# Autodesk Inventor assembly: Structure
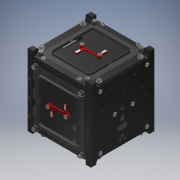
[picture p0: Inventor's stored thumbnail of the model, 180x180]
Saved by Autodesk Inventor 2018 (Build 220112000, 112)
## iProperties
Created: 2019-03-30
Part Number: Structure
Document SubType Name: Assembly
Designer: Bradley
Author: Bradley
## Documents named in this file (17)
- C:\Users\Bradley\Documents\GitHub\CougSat1-Hardware\CougSat1-Structure\CADModel\Imported\Structure.iam
- C:\Users\Bradley\Documents\GitHub\CougSat1-Hardware\CougSat1-Structure\CADModel\Imported\Structure_+X.ipt
- C:\Users\Bradley\Documents\GitHub\CougSat1-Hardware\CougSat1-Structure\CADModel\Imported\Structure_-X.ipt
- C:\Users\Bradley\Documents\GitHub\CougSat1-Hardware\CougSat1-Structure\CADModel\Imported\Structure_+Z.ipt
- C:\Users\Bradley\Documents\GitHub\CougSat1-Hardware\CougSat1-Structure\CADModel\Imported\Structure_Y.ipt
- C:\Users\Bradley\Documents\GitHub\CougSat1-Hardware\CougSat1-Structure\CADModel\Imported\Structure_-Z.ipt
- C:\Users\Bradley\Documents\GitHub\CougSat1-Hardware\CougSat1-Structure\CADModel\Imported\Structure_SolarPanelHeatsink.ipt
- C:\Users\Bradley\Documents\GitHub\CougSat1-Hardware\CougSat1-Structure\CADModel\Imported\Structure_MagnetorquerForm.ipt
- C:\Users\Bradley\Documents\GitHub\Resources\SupplierDocuments\48 - Hardware\48-0361\48-0361.ipt
- C:\Users\Bradley\Documents\GitHub\Resources\SupplierDocuments\48 - Hardware\48-0340\48-0340.ipt
- C:\Users\Bradley\Documents\GitHub\Resources\SupplierDocuments\48 - Hardware\48-0350\48-0350.ipt
- C:\Users\Bradley\Documents\GitHub\Resources\SupplierDocuments\48 - Hardware\48-0300\48-0300.ipt
- C:\Users\Bradley\Documents\GitHub\Resources\SupplierDocuments\48 - Hardware\48-0001\48-0001.ipt
- C:\Users\Bradley\Documents\GitHub\Resources\SupplierDocuments\48 - Hardware\48-0381\48-0381.ipt
- C:\Users\Bradley\Documents\GitHub\Resources\SupplierDocuments\48 - Hardware\48-0362\48-0362.ipt
- C:\Users\Bradley\Documents\GitHub\Resources\SupplierDocuments\48 - Hardware\48-03A1\48-03A1.ipt
- C:\Users\Bradley\Documents\GitHub\Resources\SupplierDocuments\49 - Electromechanical\49-0006\49-0006.ipt
## Components (81 placed, 16 different names)
1. 49-0006:3 — Mate:6, Flush:1, Flush:2
2. 49-0006:2 — Mate:4, Flush:3
3. 49-0006:1 — Mate:5, Flush:2, Flush:3
4. 48-0001:1 — Insert:27
5. 48-0001:2 — Insert:28
6. 48-0300:1 — Insert:29, Insert:30
7. 48-0300:10 — Insert:42
8. 48-0300:11 — Insert:38
9. 48-0300:12 — Insert:54
10. 48-0300:2 — Insert:53
11. 48-0300:3 — Insert:51
12. 48-0300:4 — Insert:52
13. 48-0300:5 — Insert:83, Insert:87
14. 48-0300:6 — Insert:84, Insert:88
15. 48-0300:7 — Insert:85, Insert:90
16. 48-0300:8 — Insert:86, Insert:89
17. 48-0300:9 — Insert:41
18. 48-0340:1 — Insert:77
19. 48-0340:10 — Insert:90
20. 48-0340:2 — Insert:89
21. 48-0340:3 — Insert:78
22. 48-0340:4 — Insert:79
23. 48-0340:5 — Insert:80
24. 48-0340:6 — Insert:81
25. 48-0340:7 — Insert:82
26. 48-0340:8 — Insert:87
27. 48-0340:9 — Insert:88
28. 48-0350:1 — Insert:43
29. 48-0350:2 — Insert:44
30. 48-0350:3 — Insert:45
31. 48-0350:4 — Insert:46
32. 48-0350:5 — Insert:58
33. 48-0350:6 — Insert:57
34. 48-0350:7 — Insert:55
35. 48-0350:8 — Insert:56
36. 48-0362:1 — Insert:91
37. 48-0362:2 — Insert:92
38. 48-0362:3 — Insert:94
39. 48-0362:4 — Insert:93
40. 48-0361:1 — Insert:29
41. 48-0361:2
42. 48-0361:3
43. 48-0361:4
44. 48-0361:5
45. 48-0361:6
46. 48-0361:7
47. 48-0361:8
48. 48-0381:1 — Insert:59
49. 48-0381:18 — Insert:75
50. 48-0381:2 — Insert:60
51. 48-0381:3 — Insert:63
52. 48-0381:4 — Insert:64
53. 48-0381:5 — Insert:61
54. 48-0381:6 — Insert:62
55. 48-0381:7 — Insert:65
56. 48-0381:8 — Insert:66
57. 48-0381:9 — Insert:67
58. 48-0381:10 — Insert:68
59. 48-0381:11 — Insert:69
60. 48-0381:12 — Insert:70
61. 48-0381:13 — Insert:71
62. 48-0381:14 — Insert:72
63. 48-0381:15 — Insert:74
64. 48-0381:16 — Insert:73
65. 48-0381:17 — Insert:76
66. 48-03A1:1 — Insert:95
67. 48-03A1:2 — Insert:96
68. Structure_+X:1 — Mate:1, Mate:2, Insert:1, Insert:2, Mate:3, Insert:9, Insert:10, Insert:27, Insert:77, Insert:78, Insert:79, Insert:80, Insert:81, Insert:82
69. Structure_+Z:1 — Insert:1, Insert:2, Insert:3, Insert:4, Insert:5, Insert:6, Insert:7, Insert:8, Insert:13, Insert:14, Insert:23, Insert:24, Insert:30, Insert:38, Insert:41, Insert:42, Insert:43, Insert:44, Insert:45, Insert:46
70. Structure_-X:1 — Insert:7, Insert:8, Insert:17, Insert:18, Insert:21, Insert:22, Insert:28, Mate:4, Mate:5, Mate:6, Flush:1
71. Structure_-Z:1 — Insert:9, Insert:10, Insert:51, Insert:52, Insert:53, Insert:54, Insert:55, Insert:56, Insert:57, Insert:58, Insert:83, Insert:84, Insert:85, Insert:86
72. Structure_MagnetorquerForm:1 — Insert:19, Insert:20, Insert:59, Insert:60, Insert:63, Insert:64
73. Structure_MagnetorquerForm:2 — Insert:21, Insert:22, Insert:91, Insert:92, Insert:93, Insert:94
74. Structure_MagnetorquerForm:3 — Insert:23, Insert:24, Insert:71, Insert:72, Insert:75, Insert:76
75. Structure_MagnetorquerForm:4 — Insert:25, Insert:26, Insert:65, Insert:66, Insert:69, Insert:70
76. Structure_SolarPanelHeatsink:1 — Insert:13, Insert:14, Insert:73, Insert:74
77. Structure_SolarPanelHeatsink:2 — Insert:11, Insert:12, Insert:61, Insert:62
78. Structure_SolarPanelHeatsink:3 — Insert:17, Insert:18, Insert:95, Insert:96
79. Structure_SolarPanelHeatsink:4 — Insert:15, Insert:16, Insert:67, Insert:68
80. Structure_Y:1 — Insert:3, Insert:4, Insert:11, Insert:12, Insert:19, Insert:20
81. Structure_Y:2 — Insert:5, Insert:6, Insert:15, Insert:16, Insert:25, Insert:26
## Relationships (99: Insert 90, Mate 6, Flush 3)
- Mate:1 (50 mm): Structure_+X:1
- Mate:2 (-49 mm): Structure_+X:1
- Insert:1: Structure_+X:1 ↔ Structure_+Z:1
- Insert:2: Structure_+X:1 ↔ Structure_+Z:1
- Insert:3: Structure_+Z:1 ↔ Structure_Y:1
- Insert:4: Structure_+Z:1 ↔ Structure_Y:1
- Insert:5: Structure_+Z:1 ↔ Structure_Y:2
- Insert:6: Structure_+Z:1 ↔ Structure_Y:2
- Insert:7: Structure_+Z:1 ↔ Structure_-X:1
- Insert:8: Structure_+Z:1 ↔ Structure_-X:1
- Mate:3 (50 mm): Structure_+X:1
- Insert:9: Structure_+X:1 ↔ Structure_-Z:1
- Insert:10: Structure_+X:1 ↔ Structure_-Z:1
- Insert:11: Structure_SolarPanelHeatsink:2 ↔ Structure_Y:1
- Insert:12: Structure_SolarPanelHeatsink:2 ↔ Structure_Y:1
- Insert:13: Structure_+Z:1 ↔ Structure_SolarPanelHeatsink:1
- Insert:14: Structure_+Z:1 ↔ Structure_SolarPanelHeatsink:1
- Insert:15: Structure_SolarPanelHeatsink:4 ↔ Structure_Y:2
- Insert:16: Structure_SolarPanelHeatsink:4 ↔ Structure_Y:2
- Insert:17: Structure_-X:1 ↔ Structure_SolarPanelHeatsink:3
- Insert:18: Structure_-X:1 ↔ Structure_SolarPanelHeatsink:3
- Insert:19: Structure_MagnetorquerForm:1 ↔ Structure_Y:1
- Insert:20: Structure_MagnetorquerForm:1 ↔ Structure_Y:1
- Insert:21: Structure_-X:1 ↔ Structure_MagnetorquerForm:2
- Insert:22: Structure_-X:1 ↔ Structure_MagnetorquerForm:2
- Insert:23: Structure_+Z:1 ↔ Structure_MagnetorquerForm:3
- Insert:24: Structure_+Z:1 ↔ Structure_MagnetorquerForm:3
- Insert:25: Structure_MagnetorquerForm:4 ↔ Structure_Y:2
- Insert:26: Structure_MagnetorquerForm:4 ↔ Structure_Y:2
- Insert:27: 48-0001:1 ↔ Structure_+X:1
- Insert:28: 48-0001:2 ↔ Structure_-X:1
- Insert:29: 48-0300:1 ↔ 48-0361:1
- Insert:30: 48-0300:1 ↔ Structure_+Z:1
- [Insert]: 48-0300:9 ↔ 48-0361:5
- [Insert]: 48-0300:10 ↔ 48-0361:6
- [Insert]: 48-0300:11 ↔ 48-0361:7
- Insert:38: 48-0300:11 ↔ Structure_+Z:1
- Insert:41: 48-0300:9 ↔ Structure_+Z:1
- Insert:42: 48-0300:10 ↔ Structure_+Z:1
- Insert:43: 48-0350:1 ↔ Structure_+Z:1
- Insert:44: 48-0350:2 ↔ Structure_+Z:1
- Insert:45: 48-0350:3 ↔ Structure_+Z:1
- Insert:46: 48-0350:4 ↔ Structure_+Z:1
- [Insert]: 48-0300:12 ↔ 48-0361:8
- [Insert]: 48-0300:2 ↔ 48-0361:2
- [Insert]: 48-0300:3 ↔ 48-0361:3
- [Insert]: 48-0300:4 ↔ 48-0361:4
- Insert:51: 48-0300:3 ↔ Structure_-Z:1
- Insert:52: 48-0300:4 ↔ Structure_-Z:1
- Insert:53: 48-0300:2 ↔ Structure_-Z:1
- Insert:54: 48-0300:12 ↔ Structure_-Z:1
- Insert:55: 48-0350:7 ↔ Structure_-Z:1
- Insert:56: 48-0350:8 ↔ Structure_-Z:1
- Insert:57: 48-0350:6 ↔ Structure_-Z:1
- Insert:58: 48-0350:5 ↔ Structure_-Z:1
- Insert:59 (1 mm): 48-0381:1 ↔ Structure_MagnetorquerForm:1
- Insert:60 (1 mm): 48-0381:2 ↔ Structure_MagnetorquerForm:1
- Insert:61 (1 mm): 48-0381:5 ↔ Structure_SolarPanelHeatsink:2
- Insert:62 (1 mm): 48-0381:6 ↔ Structure_SolarPanelHeatsink:2
- Insert:63 (1 mm): 48-0381:3 ↔ Structure_MagnetorquerForm:1
- Insert:64 (1 mm): 48-0381:4 ↔ Structure_MagnetorquerForm:1
- Insert:65 (1 mm): 48-0381:7 ↔ Structure_MagnetorquerForm:4
- Insert:66 (1 mm): 48-0381:8 ↔ Structure_MagnetorquerForm:4
- Insert:67 (1 mm): 48-0381:9 ↔ Structure_SolarPanelHeatsink:4
- Insert:68 (1 mm): 48-0381:10 ↔ Structure_SolarPanelHeatsink:4
- Insert:69 (1 mm): 48-0381:11 ↔ Structure_MagnetorquerForm:4
- Insert:70 (1 mm): 48-0381:12 ↔ Structure_MagnetorquerForm:4
- Insert:71 (1 mm): 48-0381:13 ↔ Structure_MagnetorquerForm:3
- Insert:72 (1 mm): 48-0381:14 ↔ Structure_MagnetorquerForm:3
- Insert:73 (1 mm): 48-0381:16 ↔ Structure_SolarPanelHeatsink:1
- Insert:74 (1 mm): 48-0381:15 ↔ Structure_SolarPanelHeatsink:1
- Insert:75 (1 mm): 48-0381:18 ↔ Structure_MagnetorquerForm:3
- Insert:76 (1 mm): 48-0381:17 ↔ Structure_MagnetorquerForm:3
- Insert:77 (1 mm): 48-0340:1 ↔ Structure_+X:1
- Insert:78 (1 mm): 48-0340:3 ↔ Structure_+X:1
- Insert:79 (1 mm): 48-0340:4 ↔ Structure_+X:1
- Insert:80 (1 mm): 48-0340:5 ↔ Structure_+X:1
- Insert:81 (1 mm): 48-0340:6 ↔ Structure_+X:1
- Insert:82 (1 mm): 48-0340:7 ↔ Structure_+X:1
- Insert:83: 48-0300:5 ↔ Structure_-Z:1
- Insert:84: 48-0300:6 ↔ Structure_-Z:1
- Insert:85: 48-0300:7 ↔ Structure_-Z:1
- Insert:86: 48-0300:8 ↔ Structure_-Z:1
- Insert:87 (1 mm): 48-0300:5 ↔ 48-0340:8
- Insert:88 (1 mm): 48-0300:6 ↔ 48-0340:9
- Insert:89 (1 mm): 48-0300:8 ↔ 48-0340:2
- Insert:90 (1 mm): 48-0300:7 ↔ 48-0340:10
- Insert:91 (1 mm): 48-0362:1 ↔ Structure_MagnetorquerForm:2
- Insert:92 (1 mm): 48-0362:2 ↔ Structure_MagnetorquerForm:2
- Insert:93 (1 mm): 48-0362:4 ↔ Structure_MagnetorquerForm:2
- Insert:94 (1 mm): 48-0362:3 ↔ Structure_MagnetorquerForm:2
- Insert:95 (1 mm): 48-03A1:1 ↔ Structure_SolarPanelHeatsink:3
- Insert:96 (1 mm): 48-03A1:2 ↔ Structure_SolarPanelHeatsink:3
- Mate:4: 49-0006:2 ↔ Structure_-X:1
- Mate:5: 49-0006:1 ↔ Structure_-X:1
- Mate:6: 49-0006:3 ↔ Structure_-X:1
- Flush:1 (14.2 mm): 49-0006:3 ↔ Structure_-X:1
- Flush:2: 49-0006:3 ↔ 49-0006:1
- Flush:3: 49-0006:2 ↔ 49-0006:1
## Named parameters: d36_d32 = 0 mm, d37_d32 = 0 mm, d40_d32 = 0 mm, d52_d32 = 0 mm, d53_d32 = 0 mm, d54_d32 = 0 mm, d55_d32 = 0 mm, SolarPanelThickness = 1 mm, PXThickness = 1 mm, NZThickness = 1 mm
